# Autodesk Inventor assembly: Bending_machine_assembly
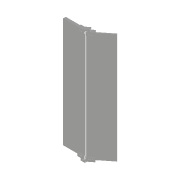
[picture p0: Inventor's stored thumbnail of the model, 180x180]
Saved by Autodesk Inventor 2022 (Build 260153000, 153)
## iProperties
Created: 2022-07-29
Part Number: Bending_machine_assembly
Document SubType Name: Assembly
Designer: dell
Author: dell
## Documents named in this file (5)
- D:\xxxx\Uni\Part IV\MECHENG_700\Part_IV_project_CAD\Bird_skeleton_prototypes\Wing_drone_V1\Bird_wing_V2\Bending_machine\Bending_machine_assembly.iam
- D:\xxxx\Uni\Part IV\MECHENG_700\Part_IV_project_CAD\Bird_skeleton_prototypes\Wing_drone_V1\Bird_wing_V2\Bending_machine\Bending_hinge.ipt
- D:\xxxx\Uni\Part IV\MECHENG_700\Part_IV_project_CAD\Bird_skeleton_prototypes\Wing_drone_V1\Bird_wing_V2\Bending_machine\Bending_plate.ipt
- D:\xxxx\Uni\Part IV\MECHENG_700\Part_IV_project_CAD\Bird_skeleton_prototypes\Wing_drone_V1\Bird_wing_V2\Bending_machine\Bending_hinge_p2.ipt
- D:\xxxx\Uni\Part IV\MECHENG_700\Part_IV_project_CAD\Bird_skeleton_prototypes\Wing_drone_V1\Bird_wing_V2\Bending_machine\Bending_plate_p2.ipt
## Components (7 placed, 4 different names)
1. Bending_hinge:1 — Mate:1, Mate:2, Mate:3, Mate:7, Mate:8
2. Bending_plate:1 — Mate:1, Mate:2, Mate:3, Mate:9, Mate:10, Mate:11, Mate:15
3. Bending_plate:4 — Mate:4, Mate:5, Mate:6, Mate:12, Mate:13, Mate:14
4. Bending_hinge_p2:1 — Mate:4, Mate:5, Mate:6, Mate:7, Mate:8
5. Bending_hinge_p2:2 — Mate:9, Mate:10, Mate:11
6. Bending_hinge:2 — Mate:12, Mate:13, Mate:14
7. Bending_plate_p2:1 — Mate:15
## Relationships (15: Mate 15)
- Mate:1: Bending_hinge:1 ↔ Bending_plate:1
- Mate:2: Bending_hinge:1 ↔ Bending_plate:1
- Mate:3 (0.05 mm): Bending_hinge:1 ↔ Bending_plate:1
- Mate:4: Bending_plate:4 ↔ Bending_hinge_p2:1
- Mate:5: Bending_plate:4 ↔ Bending_hinge_p2:1
- Mate:6 (0.05 mm): Bending_plate:4 ↔ Bending_hinge_p2:1
- Mate:7: Bending_hinge:1 ↔ Bending_hinge_p2:1
- Mate:8: Bending_hinge:1 ↔ Bending_hinge_p2:1
- Mate:9: Bending_plate:1 ↔ Bending_hinge_p2:2
- Mate:10: Bending_plate:1 ↔ Bending_hinge_p2:2
- Mate:11 (0.05 mm): Bending_plate:1 ↔ Bending_hinge_p2:2
- Mate:12: Bending_plate:4 ↔ Bending_hinge:2
- Mate:13: Bending_plate:4 ↔ Bending_hinge:2
- Mate:14 (0.05 mm): Bending_plate:4 ↔ Bending_hinge:2
- Mate:15: Bending_plate:1 ↔ Bending_plate_p2:1
